# Autodesk Inventor assembly: Leg Assembly
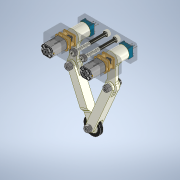
[picture p0: Inventor's stored thumbnail of the model, 180x180]
Saved by Autodesk Inventor 2022 (Build 260153000, 153)
## iProperties
Created: 2021-11-22
Part Number: Leg Assembly
Document SubType Name: Assembly
Designer: JK
Author: JK
## Documents named in this file (14)
- C:\Users\JK\Documents\Inventor\N20 Leg Actuator\CADfiles\Leg Assembly (small bearing).iam
- C:\Users\JK\Documents\Inventor\N20 Leg Actuator\CADfiles\Brushed DC Motor v8.iam
- C:\Users\JK\Documents\Inventor\N20 Leg Actuator\CADfiles\Base.ipt
- C:\Users\JK\Documents\Inventor\N20 Leg Actuator\CADfiles\Potenciometro10K.iam
- C:\Users\JK\Documents\Inventor\N20 Leg Actuator\CADfiles\PotHolder.ipt
- C:\Users\JK\Documents\Inventor\N20 Leg Actuator\CADfiles\Rubberfoot.ipt
- C:\Users\JK\Documents\Inventor\N20 Leg Actuator\CADfiles\M3 Locknut.ipt
- C:\Users\JK\Documents\Inventor\N20 Leg Actuator\CADfiles\m3x35.ipt
- C:\Users\JK\Documents\Inventor\N20 Leg Actuator\CADfiles\M3Nut.ipt
- C:\Users\JK\Documents\Inventor\N20 Leg Actuator\CADfiles\LinkA SB.ipt
- C:\Users\JK\Documents\Inventor\N20 Leg Actuator\CADfiles\LinkB SB.ipt
- C:\Users\JK\Documents\Inventor\N20 Leg Actuator\CADfiles\LinkC SB.ipt
- C:\Users\JK\Documents\Inventor\N20 Leg Actuator\CADfiles\683zz.ipt
- C:\Users\JK\Documents\Inventor\N20 Leg Actuator\CADfiles\M3x12SocketBolt.ipt
## Components (24 placed, 13 different names)
1. Brushed DC Motor v8:1 [sub-assembly] — Coincidencia:2, Coincidencia:3, Ángulo:1, Coincidencia:8
2. Brushed DC Motor v8:2 [sub-assembly] — Coincidencia:4, Ángulo:2, Coincidencia:5, Coincidencia:6, Coincidencia:7, Coincidencia:10
3. Base:1 — Coincidencia:2, Coincidencia:3, Ángulo:1, Coincidencia:4, Ángulo:2, Coincidencia:5, Ángulo:4, Ángulo:5, Coincidencia:14, Coincidencia:36, Ángulo:7, Coincidencia:42
4. LinkA SB:1 — Coincidencia:6, Coincidencia:7, Nivelación:2, Coincidencia:9, Coincidencia:10, Coincidencia:44, Nivelación:20, Coincidencia:52, Coincidencia:55
5. LinkA SB:2 — Coincidencia:8, Nivelación:2, Coincidencia:12, Coincidencia:47, Nivelación:21, Coincidencia:50, Coincidencia:53
6. Potenciometro10K:1 [sub-assembly] — Coincidencia:9, Nivelación:4, Ángulo:3, Ángulo:4, Nivelación:5
7. Potenciometro10K:2 [sub-assembly] — Nivelación:4, Coincidencia:12, Ángulo:3
8. PotHolder:1 — Ángulo:5, Coincidencia:14, Nivelación:5, Coincidencia:36, Coincidencia:37, Coincidencia:38, Coincidencia:39
9. LinkB SB:1 — Coincidencia:20, Nivelación:8, Coincidencia:30, Coincidencia:48, Coincidencia:52, Coincidencia:54, Coincidencia:57
10. LinkC SB:1 — Coincidencia:20, Nivelación:8, Coincidencia:23, Nivelación:19, Coincidencia:51, Coincidencia:53, Coincidencia:58, Nivelación:24, Ángulo:8
11. Rubberfoot:1 — Coincidencia:23, Nivelación:19, Ángulo:8
12. M3 Locknut:1 — Nivelación:13, Coincidencia:56
13. M3 Locknut:2 — Nivelación:13, Nivelación:14, Coincidencia:57
14. M3 Locknut:3 — Nivelación:14, Coincidencia:30, Coincidencia:59
15. m3x35:1 — Coincidencia:37, Nivelación:17, Coincidencia:39, Coincidencia:40
16. m3x35:2 — Coincidencia:38, Nivelación:17, Coincidencia:41
17. M3Nut:1 — Coincidencia:40, Ángulo:6, Ángulo:7, Nivelación:18, Coincidencia:42
18. M3Nut:2 — Coincidencia:41, Ángulo:6, Nivelación:18
19. 683zz:1 — Coincidencia:44, Nivelación:20, Coincidencia:48
20. 683zz:2 — Coincidencia:47, Nivelación:21
21. 683zz:3 — Coincidencia:58, Nivelación:24
22. M3x12SocketBolt:1 — Coincidencia:50, Nivelación:23, Coincidencia:56
23. M3x12SocketBolt:2 — Nivelación:22, Coincidencia:54, Coincidencia:55, Nivelación:23
24. M3x12SocketBolt:3 — Coincidencia:51, Nivelación:22, Coincidencia:59
## Relationships (56: Mate 34, Flush 14, Angle 8)
- Coincidencia:2 [Mate]: Brushed DC Motor v8:1 ↔ Base:1
- Coincidencia:3 [Mate]: Brushed DC Motor v8:1 ↔ Base:1
- Ángulo:1 [Angle] (0 deg): Brushed DC Motor v8:1 ↔ Base:1
- Coincidencia:4 [Mate]: Brushed DC Motor v8:2 ↔ Base:1
- Ángulo:2 [Angle] (0 deg): Brushed DC Motor v8:2 ↔ Base:1
- Coincidencia:5 [Mate]: Brushed DC Motor v8:2 ↔ Base:1
- Coincidencia:6 [Mate]: Brushed DC Motor v8:2 ↔ LinkA SB:1
- Coincidencia:7 [Mate]: Brushed DC Motor v8:2 ↔ LinkA SB:1
- Coincidencia:8 [Mate]: Brushed DC Motor v8:1 ↔ LinkA SB:2
- Nivelación:2 [Flush]: LinkA SB:1 ↔ LinkA SB:2
- Coincidencia:9 [Mate]: LinkA SB:1 ↔ Potenciometro10K:1
- Coincidencia:10 [Mate]: Brushed DC Motor v8:2 ↔ LinkA SB:1
- Nivelación:4 [Flush]: Potenciometro10K:1 ↔ Potenciometro10K:2
- Coincidencia:12 [Mate]: LinkA SB:2 ↔ Potenciometro10K:2
- Ángulo:3 [Angle] (0 deg): Potenciometro10K:1 ↔ Potenciometro10K:2
- Ángulo:4 [Angle] (0 deg): Base:1 ↔ Potenciometro10K:1
- Ángulo:5 [Angle] (0 deg): Base:1 ↔ PotHolder:1
- Coincidencia:14 [Mate]: Base:1 ↔ PotHolder:1
- Nivelación:5 [Flush]: Potenciometro10K:1 ↔ PotHolder:1
- Coincidencia:20 [Mate]: LinkB SB:1 ↔ LinkC SB:1
- Nivelación:8 [Flush]: LinkB SB:1 ↔ LinkC SB:1
- Coincidencia:23 [Mate]: LinkC SB:1 ↔ Rubberfoot:1
- Nivelación:13 [Flush]: M3 Locknut:1 ↔ M3 Locknut:2
- Nivelación:14 [Flush]: M3 Locknut:2 ↔ M3 Locknut:3
- Coincidencia:30 [Mate]: LinkB SB:1 ↔ M3 Locknut:3
- Coincidencia:36 [Mate]: Base:1 ↔ PotHolder:1
- Coincidencia:37 [Mate]: PotHolder:1 ↔ m3x35:1
- Coincidencia:38 [Mate]: PotHolder:1 ↔ m3x35:2
- Nivelación:17 [Flush]: m3x35:1 ↔ m3x35:2
- Coincidencia:39 [Mate]: PotHolder:1 ↔ m3x35:1
- Coincidencia:40 [Mate]: m3x35:1 ↔ M3Nut:1
- Coincidencia:41 [Mate]: m3x35:2 ↔ M3Nut:2
- Ángulo:6 [Angle] (0 deg): M3Nut:1 ↔ M3Nut:2
- Ángulo:7 [Angle] (0 deg): Base:1 ↔ M3Nut:1
- Nivelación:18 [Flush]: M3Nut:1 ↔ M3Nut:2
- Coincidencia:42 [Mate]: Base:1 ↔ M3Nut:1
- Nivelación:19 [Flush]: LinkC SB:1 ↔ Rubberfoot:1
- Coincidencia:44 [Mate]: LinkA SB:1 ↔ 683zz:1
- Nivelación:20 [Flush]: LinkA SB:1 ↔ 683zz:1
- Coincidencia:47 [Mate]: LinkA SB:2 ↔ 683zz:2
- Nivelación:21 [Flush]: LinkA SB:2 ↔ 683zz:2
- Coincidencia:48 [Mate] (0.1 mm): LinkB SB:1 ↔ 683zz:1
- Coincidencia:50 [Mate]: LinkA SB:2 ↔ M3x12SocketBolt:1
- Coincidencia:51 [Mate]: LinkC SB:1 ↔ M3x12SocketBolt:3
- Nivelación:22 [Flush]: M3x12SocketBolt:2 ↔ M3x12SocketBolt:3
- Coincidencia:52 [Mate]: LinkA SB:1 ↔ LinkB SB:1
- Coincidencia:53 [Mate]: LinkA SB:2 ↔ LinkC SB:1
- Coincidencia:54 [Mate]: LinkB SB:1 ↔ M3x12SocketBolt:2
- Coincidencia:55 [Mate]: LinkA SB:1 ↔ M3x12SocketBolt:2
- Nivelación:23 [Flush]: M3x12SocketBolt:1 ↔ M3x12SocketBolt:2
- Coincidencia:56 [Mate]: M3 Locknut:1 ↔ M3x12SocketBolt:1
- Coincidencia:57 [Mate]: LinkB SB:1 ↔ M3 Locknut:2
- Coincidencia:58 [Mate]: LinkC SB:1 ↔ 683zz:3
- Nivelación:24 [Flush]: LinkC SB:1 ↔ 683zz:3
- Coincidencia:59 [Mate]: M3 Locknut:3 ↔ M3x12SocketBolt:3
- Ángulo:8 [Angle] (180 deg): LinkC SB:1 ↔ Rubberfoot:1
